# Autodesk Inventor assembly: intake
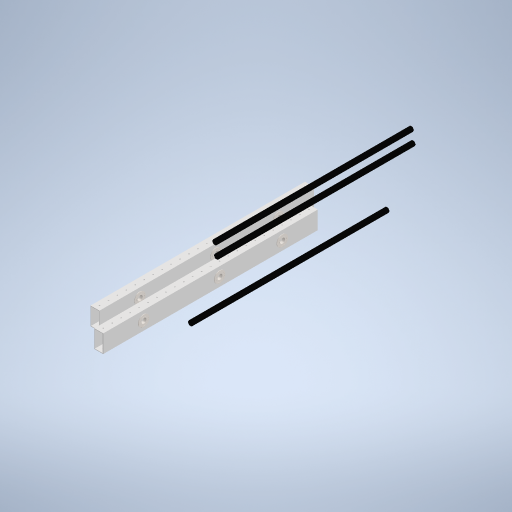
[picture p0: Inventor's stored thumbnail of the model, 512x512]
Saved by Autodesk Inventor 2023.2 (Build 272271000, 271)
## iProperties
Created: 2023-03-17
Part Number: intake
Document SubType Name: Assembly
Designer: matth
Author: matth
## Documents named in this file (4)
- D:\CAD\2023 T3\Intake\intake.iam
- C:\Users\matth\Documents\GitHub\CAD\Stock\Versa System\VersaFrame.ipt
- C:\Users\matth\Documents\GitHub\CAD\Stock\ThunderHex\Flanged Bearing.ipt
- D:\CAD\2023 T3\Intake\intake hex.ipt
## Components (17 placed, 3 different names)
1. VersaFrame:1 — Insert:1, Insert:2, Insert:3, Insert:9, Insert:11, Insert:12
2. VersaFrame:2 — Insert:4, Insert:5, Insert:6, Insert:7, Insert:8, Insert:10
3. Flanged Bearing:1 — Insert:1
4. Flanged Bearing:2 — Insert:11
5. Flanged Bearing:3 — Insert:8
6. Flanged Bearing:4 — Insert:6
7. Flanged Bearing:5 — Insert:12
8. Flanged Bearing:6 — Insert:9
9. Flanged Bearing:7 — Insert:7
10. Flanged Bearing:8 — Insert:3
11. Flanged Bearing:9 — Insert:10
12. Flanged Bearing:10 — Insert:2
13. Flanged Bearing:11 — Insert:4
14. Flanged Bearing:12 — Insert:5
15. intake hex:1
16. intake hex:2
17. intake hex:3
## Relationships (12: Insert 12)
- Insert:1: VersaFrame:1 ↔ Flanged Bearing:1
- Insert:2: VersaFrame:1 ↔ Flanged Bearing:10
- Insert:3: VersaFrame:1 ↔ Flanged Bearing:8
- Insert:4: VersaFrame:2 ↔ Flanged Bearing:11
- Insert:5: VersaFrame:2 ↔ Flanged Bearing:12
- Insert:6: VersaFrame:2 ↔ Flanged Bearing:4
- Insert:7: VersaFrame:2 ↔ Flanged Bearing:7
- Insert:8: VersaFrame:2 ↔ Flanged Bearing:3
- Insert:9: VersaFrame:1 ↔ Flanged Bearing:6
- Insert:10: VersaFrame:2 ↔ Flanged Bearing:9
- Insert:11: VersaFrame:1 ↔ Flanged Bearing:2
- Insert:12: VersaFrame:1 ↔ Flanged Bearing:5
